# Autodesk Inventor assembly: 00_XY_stage-CHUO_SEIKI_LD-647-R1
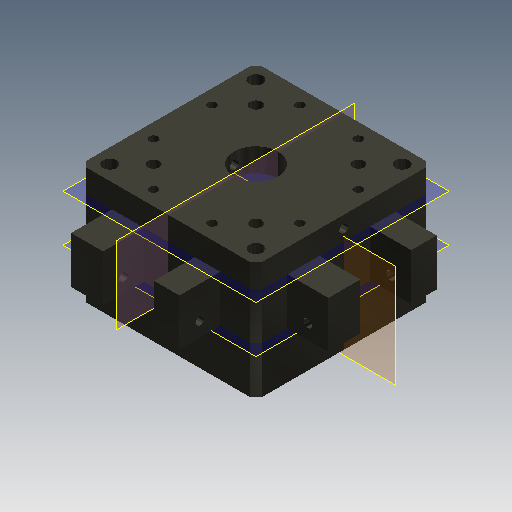
[picture p0: Inventor's stored thumbnail of the model, 512x512]
Saved by Autodesk Inventor 2019.4 (Build 234330000, 330)
## iProperties
Created: 2019-05-02
Part Number: 00_XY_stage-CHUO_SEIKI_LD-647-R1
Document SubType Name: Assembly
Designer: diederichbenedict
Author: diederichbenedict
## Documents named in this file (4)
- C:\Users\diederichbenedict\Dropbox\Dokumente\Promotion\PROJECTS\UC2\02_CAD\INVENTOR\uc2_v3\cellstrom\00_XY_stage-CHUO_SEIKI_LD-647-R1.iam
- C:\Users\diederichbenedict\Dropbox\Dokumente\Promotion\PROJECTS\UC2\02_CAD\INVENTOR\uc2_v3\cellstrom\00_XY_stage-CHUO_SEIKI_LD-647-R1-Top.ipt
- C:\Users\diederichbenedict\Dropbox\Dokumente\Promotion\PROJECTS\UC2\02_CAD\INVENTOR\uc2_v3\cellstrom\00_XY_stage-CHUO_SEIKI_LD-647-R1-Middle.ipt
- C:\Users\diederichbenedict\Dropbox\Dokumente\Promotion\PROJECTS\UC2\02_CAD\INVENTOR\uc2_v3\cellstrom\00_XY_stage-CHUO_SEIKI_LD-647-R1-Bottom.ipt
## Components (3 placed, 3 different names)
1. 00_XY_stage-CHUO_SEIKI_LD-647-R1-Top:1 — Flush:1, Flush:2, Mate:1, Symmetry:1, Symmetry:2
2. 00_XY_stage-CHUO_SEIKI_LD-647-R1-Middle:1 — Flush:1, Flush:2, Flush:3, Flush:4, Mate:1, Symmetry:1, Symmetry:2, Symmetry:3
3. 00_XY_stage-CHUO_SEIKI_LD-647-R1-Bottom:1 — Flush:3, Flush:4, Symmetry:3
## Relationships (8: Flush 4, Symmetry 3, Mate 1)
- Flush:1: 00_XY_stage-CHUO_SEIKI_LD-647-R1-Top:1 ↔ 00_XY_stage-CHUO_SEIKI_LD-647-R1-Middle:1
- Flush:2: 00_XY_stage-CHUO_SEIKI_LD-647-R1-Top:1 ↔ 00_XY_stage-CHUO_SEIKI_LD-647-R1-Middle:1
- Flush:3: 00_XY_stage-CHUO_SEIKI_LD-647-R1-Middle:1 ↔ 00_XY_stage-CHUO_SEIKI_LD-647-R1-Bottom:1
- Flush:4: 00_XY_stage-CHUO_SEIKI_LD-647-R1-Middle:1 ↔ 00_XY_stage-CHUO_SEIKI_LD-647-R1-Bottom:1
- Mate:1: 00_XY_stage-CHUO_SEIKI_LD-647-R1-Top:1 ↔ 00_XY_stage-CHUO_SEIKI_LD-647-R1-Middle:1
- Symmetry:1: 00_XY_stage-CHUO_SEIKI_LD-647-R1-Top:1 ↔ 00_XY_stage-CHUO_SEIKI_LD-647-R1-Middle:1
- Symmetry:2: 00_XY_stage-CHUO_SEIKI_LD-647-R1-Top:1 ↔ 00_XY_stage-CHUO_SEIKI_LD-647-R1-Middle:1
- Symmetry:3: 00_XY_stage-CHUO_SEIKI_LD-647-R1-Middle:1 ↔ 00_XY_stage-CHUO_SEIKI_LD-647-R1-Bottom:1
